# Autodesk Inventor assembly: Chassis 2
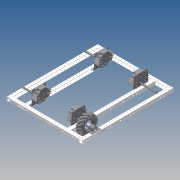
[picture p0: Inventor's stored thumbnail of the model, 180x180]
Saved by Autodesk Inventor 2014 SP1 (Build 180222100, 222)
## iProperties
Created: 2014-01-31
Part Number: Chassis 2
Document SubType Name: Assembly
Designer: Pradhan Alexander
Author: Pradhan Alexander
## Documents named in this file (9)
- \\STUCLUSTER\Shared\MHS\Technology\Holliday B\Group Projects\Robotics\CAD Team\CAD Team 2014\Chassis 2014\Chassis 2.iam
- \\STUCLUSTER\Shared\MHS\Technology\Holliday B\Group Projects\Robotics\CAD Team\CAD Team 2014\Chassis 2014\Chassis_Channel_AndyMark_am-0202-23in.ipt
- \\STUCLUSTER\Shared\MHS\Technology\Holliday B\Group Projects\Robotics\CAD Team\CAD Team 2014\Chassis 2014\Chassis_Channel_AndyMark_am-0202-28in.ipt
- \\STUCLUSTER\Shared\MHS\Technology\Holliday B\Group Projects\Robotics\CAD Team\CAD Team 2014\Chassis 2014\Chassis_Channel_AndyMark_am-0202-30in.ipt
- \\STUCLUSTER\Shared\MHS\Technology\Holliday B\Group Projects\Robotics\CAD Team\CAD Team 2014\Chassis 2014\Toughbox-mini with long shaft.iam
- \\STUCLUSTER\Shared\MHS\Technology\Holliday B\Group Projects\Robotics\CAD Team\CAD Team 2014\Chassis 2014\Bearing mount.ipt
- \\Stucluster\Home\2016\Pradhan Alexander\Inventor\Right-6-inch-HD-Mecanum-Wheel.iam
- \\STUCLUSTER\Shared\MHS\Technology\Holliday B\Group Projects\Robotics\CAD Team\CAD Team 2014\Chassis 2014\am-0077a-500 Key Hub r2.ipt
- \\STUCLUSTER\Shared\MHS\Technology\Holliday B\Group Projects\Robotics\CAD Team\CAD Team 2014\Chassis 2014\.75in Spacer.ipt
## Components (16 placed, 8 different names)
1. Chassis_Channel_AndyMark_am-0202-23in:1 — Mate:12, Flush:4, Mate:15, Angle:5
2. Chassis_Channel_AndyMark_am-0202-23in:2 — Mate:1, Angle:1, Mate:5, Flush:2, Flush:3, Mate:18, Angle:6, Mate:21, Angle:7, Mate:23, Flush:6, Mate:24, Flush:8
3. Chassis_Channel_AndyMark_am-0202-28in:1 — Mate:24, Flush:8, Flush:9, Insert:1, Insert:2, Insert:5, Insert:6
4. Chassis_Channel_AndyMark_am-0202-28in:2 — Mate:23, Flush:6, Flush:7, Insert:3, Insert:4, Insert:7, Insert:8
5. Chassis_Channel_AndyMark_am-0202-30in:1 — Mate:9, Angle:3, Flush:3, Mate:12, Flush:4, Mate:13, Angle:4
6. Chassis_Channel_AndyMark_am-0202-30in:2 — Mate:3, Angle:2, Mate:5, Flush:2, Mate:25
7. Toughbox-mini with long shaft:1 [sub-assembly] — Insert:1, Insert:2
8. Toughbox-mini with long shaft:2 [sub-assembly] — Insert:5, Insert:6
9. Toughbox-mini with long shaft:3 [sub-assembly] — Insert:7, Insert:8
10. Toughbox-mini with long shaft:4 [sub-assembly] — Insert:3, Insert:4, Mate:26, Insert:13
11. Bearing mount:1 — Mate:25
12. Right-6-inch-HD-Mecanum-Wheel:1 [sub-assembly] — Insert:9, Insert:10, Insert:11, Insert:12
13. am-0077a-500 Key Hub r2:1 — Insert:11, Insert:12, Mate:26, Insert:15
14. am-0077a-500 Key Hub r2:2 — Insert:9, Insert:10
15. .75in Spacer:1 — Insert:14, Insert:15
16. .75in Spacer:2 — Insert:13, Insert:14
## Relationships (52: Mate 21, Insert 15, Flush 9, Angle 7)
- Mate:1: Chassis_Channel_AndyMark_am-0202-23in:2
- Mate:2
- Angle:1 (0 deg): Chassis_Channel_AndyMark_am-0202-23in:2
- Mate:3: Chassis_Channel_AndyMark_am-0202-30in:2
- Mate:4
- Angle:2 (90 deg): Chassis_Channel_AndyMark_am-0202-30in:2
- Mate:5: Chassis_Channel_AndyMark_am-0202-23in:2 ↔ Chassis_Channel_AndyMark_am-0202-30in:2
- Flush:1
- Flush:2: Chassis_Channel_AndyMark_am-0202-23in:2 ↔ Chassis_Channel_AndyMark_am-0202-30in:2
- Mate:9: Chassis_Channel_AndyMark_am-0202-30in:1
- Mate:10
- Angle:3 (90 deg): Chassis_Channel_AndyMark_am-0202-30in:1
- Mate:11
- Flush:3: Chassis_Channel_AndyMark_am-0202-23in:2 ↔ Chassis_Channel_AndyMark_am-0202-30in:1
- Mate:12: Chassis_Channel_AndyMark_am-0202-23in:1 ↔ Chassis_Channel_AndyMark_am-0202-30in:1
- Flush:4: Chassis_Channel_AndyMark_am-0202-23in:1 ↔ Chassis_Channel_AndyMark_am-0202-30in:1
- Mate:13: Chassis_Channel_AndyMark_am-0202-30in:1
- Mate:14
- Angle:4 (90 deg): Chassis_Channel_AndyMark_am-0202-30in:1
- Mate:15: Chassis_Channel_AndyMark_am-0202-23in:1
- Mate:16
- Angle:5 (0 deg): Chassis_Channel_AndyMark_am-0202-23in:1
- Flush:5
- Mate:18: Chassis_Channel_AndyMark_am-0202-23in:2
- Mate:19
- Angle:6 (90 deg): Chassis_Channel_AndyMark_am-0202-23in:2
- Mate:21: Chassis_Channel_AndyMark_am-0202-23in:2
- Mate:22
- Angle:7 (90 deg): Chassis_Channel_AndyMark_am-0202-23in:2
- Mate:23: Chassis_Channel_AndyMark_am-0202-23in:2 ↔ Chassis_Channel_AndyMark_am-0202-28in:2
- Flush:6: Chassis_Channel_AndyMark_am-0202-23in:2 ↔ Chassis_Channel_AndyMark_am-0202-28in:2
- Flush:7: Chassis_Channel_AndyMark_am-0202-28in:2
- Mate:24: Chassis_Channel_AndyMark_am-0202-23in:2 ↔ Chassis_Channel_AndyMark_am-0202-28in:1
- Flush:8: Chassis_Channel_AndyMark_am-0202-23in:2 ↔ Chassis_Channel_AndyMark_am-0202-28in:1
- Flush:9: Chassis_Channel_AndyMark_am-0202-28in:1
- Insert:1: Chassis_Channel_AndyMark_am-0202-28in:1 ↔ Toughbox-mini with long shaft:1
- Insert:2: Chassis_Channel_AndyMark_am-0202-28in:1 ↔ Toughbox-mini with long shaft:1
- Insert:3: Chassis_Channel_AndyMark_am-0202-28in:2 ↔ Toughbox-mini with long shaft:4
- Insert:4: Chassis_Channel_AndyMark_am-0202-28in:2 ↔ Toughbox-mini with long shaft:4
- Insert:5: Chassis_Channel_AndyMark_am-0202-28in:1 ↔ Toughbox-mini with long shaft:2
- Insert:6: Chassis_Channel_AndyMark_am-0202-28in:1 ↔ Toughbox-mini with long shaft:2
- Insert:7: Chassis_Channel_AndyMark_am-0202-28in:2 ↔ Toughbox-mini with long shaft:3
- Insert:8: Chassis_Channel_AndyMark_am-0202-28in:2 ↔ Toughbox-mini with long shaft:3
- Mate:25: Chassis_Channel_AndyMark_am-0202-30in:2 ↔ Bearing mount:1
- Insert:9: Right-6-inch-HD-Mecanum-Wheel:1 ↔ am-0077a-500 Key Hub r2:2
- Insert:10: Right-6-inch-HD-Mecanum-Wheel:1 ↔ am-0077a-500 Key Hub r2:2
- Insert:11: Right-6-inch-HD-Mecanum-Wheel:1 ↔ am-0077a-500 Key Hub r2:1
- Insert:12: Right-6-inch-HD-Mecanum-Wheel:1 ↔ am-0077a-500 Key Hub r2:1
- Mate:26: Toughbox-mini with long shaft:4 ↔ am-0077a-500 Key Hub r2:1
- Insert:13: Toughbox-mini with long shaft:4 ↔ .75in Spacer:2
- Insert:14: .75in Spacer:1 ↔ .75in Spacer:2
- Insert:15: am-0077a-500 Key Hub r2:1 ↔ .75in Spacer:1
